# Autodesk Inventor assembly: MegahashColdStorage_V3
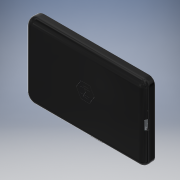
[picture p0: Inventor's stored thumbnail of the model, 180x180]
Saved by Autodesk Inventor 2017 (Build 210142000, 142)
## iProperties
Created: 2018-08-13
Part Number: MegahashColdStorage_V3
Document SubType Name: Assembly
Designer: intelsath
Author: intelsath
## Documents named in this file (9)
- C:\Users\intelsath\Documents\Inventor\Cryptowallet\MegahashColdStorage_V3.iam
- C:\Users\intelsath\Documents\Inventor\Cryptowallet\Casing for cover.ipt
- C:\Users\intelsath\Documents\Inventor\Cryptowallet\Touchcreen+Cover.ipt
- C:\Users\intelsath\Documents\Inventor\Cryptowallet\Multi-Inno_3.5in_LCD.ipt
- C:\Users\intelsath\Documents\Inventor\Cryptowallet\Assembled_PCB.iam
- C:\Users\intelsath\Documents\Inventor\Cryptowallet\Battery.ipt
- C:\Users\intelsath\Documents\Inventor\Cryptowallet\Antenna.ipt
- C:\Users\intelsath\Documents\Inventor\Cryptowallet\LED Pipe.ipt
- C:\Users\intelsath\Documents\Inventor\Cryptowallet\Button Cap.ipt
## Components (8 placed, 8 different names)
1. Casing for cover:1 — Cylindrical:1, Cylindrical:2, Cylindrical:3, Cylindrical:4, Mate:1, Mate:3, Cylindrical:5, Cylindrical:6, Cylindrical:7, Mate:7
2. Touchcreen+Cover:1 — Rigid:1, Cylindrical:1, Cylindrical:2
3. Multi-Inno_3.5in_LCD:1 — Rigid:1, Mate:8
4. Assembled_PCB:1 [sub-assembly] — Cylindrical:3, Cylindrical:4, Flush:1, Mate:2, Flush:2, Flush:3, Flush:4, Mate:6
5. Battery:1 — Flush:1, Mate:1, Mate:2, Mate:7, Mate:8
6. Antenna:1 — Mate:3, Flush:2, Flush:3
7. LED Pipe:1 — Cylindrical:5, Flush:4
8. Button Cap:1 — Cylindrical:6, Cylindrical:7, Mate:6
## Relationships (18: CylindricalJoint 7, Mate 6, Flush 4, WeldJoint 1)
- Rigid:1 [WeldJoint] (0.07 mm): Touchcreen+Cover:1 ↔ Multi-Inno_3.5in_LCD:1
- Cylindrical:1: Casing for cover:1 ↔ Touchcreen+Cover:1
- Cylindrical:2: Casing for cover:1 ↔ Touchcreen+Cover:1
- Cylindrical:3: Casing for cover:1 ↔ Assembled_PCB:1
- Cylindrical:4: Casing for cover:1 ↔ Assembled_PCB:1
- Flush:1: Assembled_PCB:1 ↔ Battery:1
- Mate:1: Casing for cover:1 ↔ Battery:1
- Mate:2: Assembled_PCB:1 ↔ Battery:1
- Mate:3: Casing for cover:1 ↔ Antenna:1
- Flush:2 (20.6 mm): Assembled_PCB:1 ↔ Antenna:1
- Flush:3 (0.5 mm): Assembled_PCB:1 ↔ Antenna:1
- Cylindrical:5: Casing for cover:1 ↔ LED Pipe:1
- Flush:4 (-4 mm): Assembled_PCB:1 ↔ LED Pipe:1
- Cylindrical:6: Casing for cover:1 ↔ Button Cap:1
- Cylindrical:7: Casing for cover:1 ↔ Button Cap:1
- Mate:6: Assembled_PCB:1 ↔ Button Cap:1
- Mate:7: Casing for cover:1 ↔ Battery:1
- Mate:8: Multi-Inno_3.5in_LCD:1 ↔ Battery:1
